# Autodesk Inventor assembly: Bottom Mold_Remote Bottom_LY
Saved by Autodesk Inventor 2016 (Build 200138000, 138)
## iProperties
Created: 2015-07-09
Part Number: Bottom Mold_Remote Bottom_LY
Document SubType Name: Assembly
Designer: Samuel Clay
Author: Samuel Clay
## Documents named in this file (2)
- Z:\turntouch\remote\enclosure\inventor\Molds\Bottom Mold_Remote Bottom_LY.iam
- Z:\turntouch\remote\enclosure\inventor\Molds\Bottom Mold_Remote Bottom_PZ.iam
## Components (1 placed, 1 different names)
1. Bottom Mold_Remote Bottom_PZ:1 [sub-assembly] — Flush:1, Flush:2, Flush:3
## Relationships (3: Flush 3)
- Flush:1: Bottom Mold_Remote Bottom_PZ:1
- Flush:2: Bottom Mold_Remote Bottom_PZ:1
- Flush:3: Bottom Mold_Remote Bottom_PZ:1
